# Autodesk Inventor assembly: Reducotora
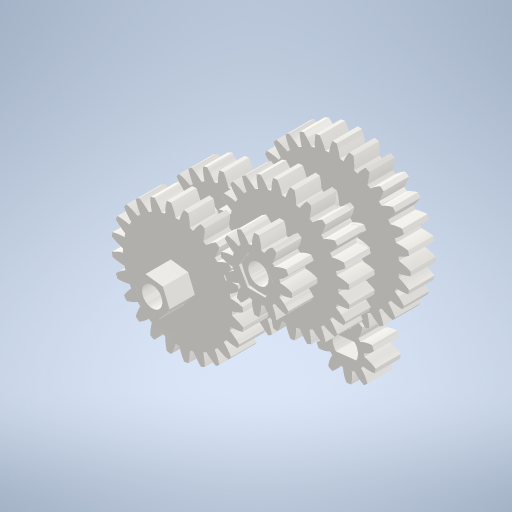
[picture p0: Inventor's stored thumbnail of the model, 512x512]
Saved by Autodesk Inventor 2023 (Build 270158000, 158)
## iProperties
Created: 2022-12-05
Part Number: Reducotora
Document SubType Name: Assembly
Designer: sergi
Author: sergi
## Documents named in this file (5)
- C:\Users\sergi\OneDrive\Escritorio\Objetos 3d\ComederoV3\Reducotora.iam
- C:\Users\sergi\OneDrive\Escritorio\Objetos 3d\ComederoV3\Reducotora\Design Accelerator\Engranajes rectos1.iam
- C:\Users\sergi\OneDrive\Escritorio\Objetos 3d\ComederoV3\Reducotora\Design Accelerator\Engranajes rectos2.iam
- C:\Users\sergi\OneDrive\Escritorio\Objetos 3d\ComederoV3\Reducotora\Design Accelerator\Engranajes rectos3.iam
- C:\Users\sergi\OneDrive\Escritorio\Objetos 3d\ComederoV3\Reducotora\Design Accelerator\Engranajes rectos4.iam
## Components (6 placed, 1 different names)
1. Engranajes rectos:1 [sub-assembly]
2. Engranajes rectos:2 [sub-assembly]
3. Engranajes rectos:3 [sub-assembly] — Coincidencia:2, Coincidencia:4, Rotación:1, Coincidencia:7
4. Engranajes rectos:4 [sub-assembly] — Coincidencia:2, Coincidencia:4, Rotación:1, Coincidencia:5, Rotación:2, Coincidencia:6, Coincidencia:9
5. Engranajes rectos:5 [sub-assembly] — Coincidencia:5, Rotación:2, Coincidencia:6, Coincidencia:7, Coincidencia:8
6. Engranajes rectos:6 [sub-assembly] — Coincidencia:8, Coincidencia:9
## Relationships (9: Mate 7, RelateRotation 2)
- Coincidencia:2 [Mate]: Engranajes rectos:3 ↔ Engranajes rectos:4
- Coincidencia:4 [Mate]: Engranajes rectos:3 ↔ Engranajes rectos:4
- Rotación:1 [RelateRotation] (0.421 ul): Engranajes rectos:3 ↔ Engranajes rectos:4
- Coincidencia:5 [Mate]: Engranajes rectos:4 ↔ Engranajes rectos:5
- Rotación:2 [RelateRotation] (1 ul): Engranajes rectos:4 ↔ Engranajes rectos:5
- Coincidencia:6 [Mate]: Engranajes rectos:4 ↔ Engranajes rectos:5
- Coincidencia:7 [Mate]: Engranajes rectos:3 ↔ Engranajes rectos:5
- Coincidencia:8 [Mate]: Engranajes rectos:5 ↔ Engranajes rectos:6
- Coincidencia:9 [Mate]: Engranajes rectos:4 ↔ Engranajes rectos:6
